# Autodesk Inventor assembly: Robot
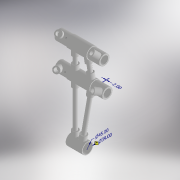
[picture p0: Inventor's stored thumbnail of the model, 180x180]
Saved by Autodesk Inventor 2021 (Build 250183000, 183)
## iProperties
Created: 2024-02-19
Part Number: Robot
Document SubType Name: Assembly
Designer: Martin
Author: Martin
## Documents named in this file (12)
- C:\Users\ASUS\OneDrive - Universidad de Antioquia\2024-1\Robótica\CAD\Robot.iam
- C:\Users\ASUS\OneDrive - Universidad de Antioquia\2024-1\Robótica\CAD\JuntaRodilla.ipt
- C:\Users\ASUS\OneDrive - Universidad de Antioquia\2024-1\Robótica\CAD\SoporteMotor.ipt
- C:\Users\ASUS\OneDrive - Universidad de Antioquia\2024-1\Robótica\CAD\Tubo1.ipt
- C:\Users\ASUS\OneDrive - Universidad de Antioquia\2024-1\Robótica\CAD\Tubo2.ipt
- C:\Users\ASUS\OneDrive - Universidad de Antioquia\2024-1\Robótica\CAD\EjeRodilla.ipt
- C:\Users\ASUS\OneDrive - Universidad de Antioquia\2024-1\Robótica\CAD\JuntaEjeCadera.ipt
- C:\Users\ASUS\OneDrive - Universidad de Antioquia\2024-1\Robótica\CAD\Tubo3.ipt
- C:\Users\ASUS\OneDrive - Universidad de Antioquia\2024-1\Robótica\CAD\Tubo4.ipt
- C:\Users\ASUS\OneDrive - Universidad de Antioquia\2024-1\Robótica\CAD\JuntaRodilla2.ipt
- C:\Users\ASUS\OneDrive - Universidad de Antioquia\2024-1\Robótica\CAD\JuntaEje2Trasero.ipt
- C:\Users\ASUS\OneDrive - Universidad de Antioquia\2024-1\Robótica\CAD\EjeRodilla2.ipt
## Components (13 placed, 11 different names)
1. JuntaRodilla:1 — Mate:5, Mate:6, Mate:7, Mate:11, Mate:12, Mate:13, Mate:14, Mate:23
2. SoporteMotor:1 — Mate:1, Mate:2, Mate:3, Mate:4
3. Tubo1:1 — Mate:1, Mate:2, Mate:5
4. Tubo2:1 — Mate:3, Mate:4, Mate:6
5. EjeRodilla:1 — Mate:7, Mate:9, Mate:10, Mate:21, Mate:22
6. JuntaEjeCadera:1 — Mate:9, Mate:10
7. Tubo3:1 — Mate:11, Mate:12, Mate:15
8. Tubo4:1 — Mate:13, Mate:14, Mate:16
9. JuntaRodilla2:1 — Mate:15, Mate:16, Mate:27, Mate:30
10. JuntaEje2Trasero:1 — Mate:25, Mate:26
11. JuntaEjeCadera:2 — Mate:21, Mate:22, Mate:23
12. EjeRodilla2:1 — Mate:25, Mate:26, Mate:27, Mate:28, Mate:29
13. JuntaEje2Trasero:2 — Mate:28, Mate:29, Mate:30
## Relationships (24: Mate 24)
- Mate:1: SoporteMotor:1 ↔ Tubo1:1
- Mate:2 (-20 mm): SoporteMotor:1 ↔ Tubo1:1
- Mate:3: SoporteMotor:1 ↔ Tubo2:1
- Mate:4 (-20 mm): SoporteMotor:1 ↔ Tubo2:1
- Mate:5: JuntaRodilla:1 ↔ Tubo1:1
- Mate:6: JuntaRodilla:1 ↔ Tubo2:1
- Mate:7: JuntaRodilla:1 ↔ EjeRodilla:1
- Mate:9: EjeRodilla:1 ↔ JuntaEjeCadera:1
- Mate:10: EjeRodilla:1 ↔ JuntaEjeCadera:1
- Mate:11: JuntaRodilla:1 ↔ Tubo3:1
- Mate:12 (-15 mm): JuntaRodilla:1 ↔ Tubo3:1
- Mate:13: JuntaRodilla:1 ↔ Tubo4:1
- Mate:14 (-15 mm): JuntaRodilla:1 ↔ Tubo4:1
- Mate:15: Tubo3:1 ↔ JuntaRodilla2:1
- Mate:16: Tubo4:1 ↔ JuntaRodilla2:1
- Mate:21: EjeRodilla:1 ↔ JuntaEjeCadera:2
- Mate:22: EjeRodilla:1 ↔ JuntaEjeCadera:2
- Mate:23: JuntaRodilla:1 ↔ JuntaEjeCadera:2
- Mate:25: JuntaEje2Trasero:1 ↔ EjeRodilla2:1
- Mate:26: JuntaEje2Trasero:1 ↔ EjeRodilla2:1
- Mate:27: JuntaRodilla2:1 ↔ EjeRodilla2:1
- Mate:28: EjeRodilla2:1 ↔ JuntaEje2Trasero:2
- Mate:29: EjeRodilla2:1 ↔ JuntaEje2Trasero:2
- Mate:30: JuntaRodilla2:1 ↔ JuntaEje2Trasero:2
